# Autodesk Inventor assembly: AssemblyFinal
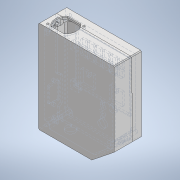
[picture p0: Inventor's stored thumbnail of the model, 180x180]
Saved by Autodesk Inventor 2020 (Build 240168000, 168)
## iProperties
Created: 2020-04-13
Part Number: AssemblyFinal
Document SubType Name: Assembly
Designer: Windooof
Author: Windooof
## Documents named in this file (3)
- C:\Users\Windooof\Documents\Inventor\Facharbeit\AssemblyFinal.iam
- C:\Users\Windooof\Documents\Inventor\Facharbeit\Case.ipt
- C:\Users\Windooof\Documents\Inventor\Facharbeit\CaseLid.ipt
## Components (2 placed, 2 different names)
1. Case:1 — Fluchtend:1, Fluchtend:2, Passend:1
2. CaseLid:1 — Fluchtend:1, Fluchtend:2, Passend:1
## Relationships (3: Flush 2, Mate 1)
- Fluchtend:1 [Flush]: Case:1 ↔ CaseLid:1
- Fluchtend:2 [Flush]: Case:1 ↔ CaseLid:1
- Passend:1 [Mate]: Case:1 ↔ CaseLid:1
